# Autodesk Inventor assembly: Rear Crossbrace
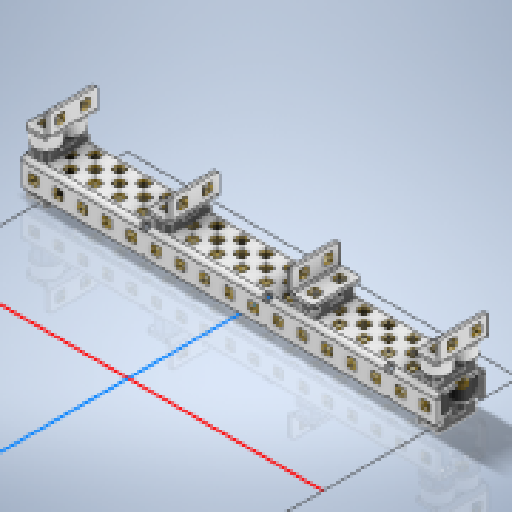
[picture p0: Inventor's stored thumbnail of the model, 512x512]
Saved by Autodesk Inventor 2026 (Build 300175000, 175)
## iProperties
Created: 2025-04-02
Part Number: Rear Crossbrace
Document SubType Name: Assembly
Designer: avere
Author: avere
## Documents named in this file (10)
- C:\Users\avere\OneDrive\Documents\VEX-CAD\V5-CAD\drivetrain\Braces\Rear Crossbrace.iam
- C:\Users\avere\OneDrive\Documents\VEX-CAD\VEX-CAD-Inventor\Structure\C Channel\Aluminum 1x2x1\Alu C 1x2x1x17.ipt
- C:\Users\avere\OneDrive\Documents\VEX-CAD\VEX-CAD-Inventor\Structure\Angle\Aluminum 1x1\Alu Angle 1x1x2.ipt
- C:\Users\avere\OneDrive\Documents\VEX-CAD\VEX-CAD-Inventor\Motion\Shaft LS\Bearing Flat - Cut.ipt
- C:\Users\avere\OneDrive\Documents\VEX-CAD\VEX-CAD-Inventor\Motion\Spacers\Spacer Nylon .375 OD\NSpacer .375 OD x .375.ipt
- C:\Users\avere\OneDrive\Documents\VEX-CAD\VEX-CAD-Inventor\Motion\Spacers\Spacer Nylon .375 OD.ipt
- C:\Users\avere\OneDrive\Documents\VEX-CAD\VEX-CAD-Inventor\Motion\Spacers\Washer Steel\SWasher .375 OD x .062500.ipt
- C:\Users\avere\OneDrive\Documents\VEX-CAD\VEX-CAD-Inventor\Motion\Spacers\Washer Steel.ipt
- C:\Users\avere\OneDrive\Documents\VEX-CAD\VEX-CAD-Inventor\Motion\Spacers\Spacer Nylon .500 OD\NSpacer White .500 OD x .250.ipt
- C:\Users\avere\OneDrive\Documents\VEX-CAD\VEX-CAD-Inventor\Motion\Spacers\Spacer Nylon .500 OD.ipt
## Components (23 placed, 6 different names)
1. Alu C 1x2x1x17:1 — Mate:1, Flush:1, Insert:1, Mate:4, Insert:12, Mate:7, Insert:22, Mate:10, Insert:30, Mate:16
2. Alu Angle 1x1x2:1 — Insert:2, Mate:3
3. Bearing Flat - Cut:1 — Insert:1, Insert:2, Mate:3, Mate:4
4. Alu Angle 1x1x2:2 — Mate:5, Insert:3, Mate:6
5. Bearing Flat - Cut:2 — Mate:5, Insert:3, Mate:6
6. Bearing Flat - Cut:3 — Insert:10, Insert:11
7. NSpacer .375 OD x .375:1 — Insert:8, Insert:10
8. SWasher .375 OD x .062500:1 — Insert:8, Insert:12
9. NSpacer .375 OD x .375:2 — Insert:9, Insert:11
10. SWasher .375 OD x .062500:2 — Insert:9, Mate:7
11. Bearing Flat - Cut:4 — Insert:13, Insert:14, Insert:17, Insert:18
12. NSpacer .375 OD x .375:3 — Insert:13, Insert:14, Insert:15, Insert:16
13. SWasher .375 OD x .062500:3 — Insert:15, Insert:16
14. NSpacer .375 OD x .375:4 — Insert:17, Insert:18, Insert:19, Insert:20
15. SWasher .375 OD x .062500:4 — Insert:19, Insert:20
16. Alu Angle 1x1x2:3 — Insert:31, Mate:17
17. Bearing Flat - Cut:5 — Insert:22, Mate:10, Insert:25, Insert:26
18. NSpacer White .500 OD x .250:1 — Insert:25, Mate:17
19. NSpacer White .500 OD x .250:2 — Insert:26, Insert:31
20. Alu Angle 1x1x2:5 — Insert:27, Mate:14, Mate:15
21. Bearing Flat - Cut:7 — Insert:27, Mate:14, Mate:15, Insert:28, Insert:29, Insert:30
22. NSpacer White .500 OD x .250:3 — Insert:28, Mate:16
23. NSpacer White .500 OD x .250:4 — Insert:29
## Relationships (41: Insert 28, Mate 12, Flush 1)
- Mate:1 (50.8 mm): Alu C 1x2x1x17:1
- Flush:1 (-107.95 mm): Alu C 1x2x1x17:1
- [Mate]: Alu Angle 1x1x2:1 ↔ Bearing Flat - Cut:1
- Insert:1: Alu C 1x2x1x17:1 ↔ Bearing Flat - Cut:1
- Insert:2: Alu Angle 1x1x2:1 ↔ Bearing Flat - Cut:1
- Mate:3: Alu Angle 1x1x2:1 ↔ Bearing Flat - Cut:1
- Mate:4: Alu C 1x2x1x17:1 ↔ Bearing Flat - Cut:1
- Mate:5: Alu Angle 1x1x2:2 ↔ Bearing Flat - Cut:2
- Insert:3: Alu Angle 1x1x2:2 ↔ Bearing Flat - Cut:2
- Mate:6: Alu Angle 1x1x2:2 ↔ Bearing Flat - Cut:2
- [Insert]: NSpacer .375 OD x .375:1 ↔ SWasher .375 OD x .062500:1
- [Insert]: Bearing Flat - Cut:3 ↔ NSpacer .375 OD x .375:1
- [Insert]: NSpacer .375 OD x .375:2 ↔ SWasher .375 OD x .062500:2
- [Insert]: Bearing Flat - Cut:3 ↔ NSpacer .375 OD x .375:2
- Insert:8: NSpacer .375 OD x .375:1 ↔ SWasher .375 OD x .062500:1
- Insert:9: NSpacer .375 OD x .375:2 ↔ SWasher .375 OD x .062500:2
- Insert:10: Bearing Flat - Cut:3 ↔ NSpacer .375 OD x .375:1
- Insert:11: Bearing Flat - Cut:3 ↔ NSpacer .375 OD x .375:2
- Insert:12: Alu C 1x2x1x17:1 ↔ SWasher .375 OD x .062500:1
- Mate:7: Alu C 1x2x1x17:1 ↔ SWasher .375 OD x .062500:2
- Insert:13: Bearing Flat - Cut:4 ↔ NSpacer .375 OD x .375:3
- Insert:14: Bearing Flat - Cut:4 ↔ NSpacer .375 OD x .375:3
- Insert:15: NSpacer .375 OD x .375:3 ↔ SWasher .375 OD x .062500:3
- Insert:16: NSpacer .375 OD x .375:3 ↔ SWasher .375 OD x .062500:3
- Insert:17: Bearing Flat - Cut:4 ↔ NSpacer .375 OD x .375:4
- Insert:18: Bearing Flat - Cut:4 ↔ NSpacer .375 OD x .375:4
- Insert:19: NSpacer .375 OD x .375:4 ↔ SWasher .375 OD x .062500:4
- Insert:20: NSpacer .375 OD x .375:4 ↔ SWasher .375 OD x .062500:4
- Insert:22: Alu C 1x2x1x17:1 ↔ Bearing Flat - Cut:5
- Mate:10: Alu C 1x2x1x17:1 ↔ Bearing Flat - Cut:5
- Insert:25: Bearing Flat - Cut:5 ↔ NSpacer White .500 OD x .250:1
- Insert:26: Bearing Flat - Cut:5 ↔ NSpacer White .500 OD x .250:2
- Insert:27 (6.35 mm): Alu Angle 1x1x2:5 ↔ Bearing Flat - Cut:7
- Mate:14: Alu Angle 1x1x2:5 ↔ Bearing Flat - Cut:7
- Mate:15: Alu Angle 1x1x2:5 ↔ Bearing Flat - Cut:7
- Insert:28: Bearing Flat - Cut:7 ↔ NSpacer White .500 OD x .250:3
- Insert:29: Bearing Flat - Cut:7 ↔ NSpacer White .500 OD x .250:4
- Insert:30: Alu C 1x2x1x17:1 ↔ Bearing Flat - Cut:7
- Mate:16: Alu C 1x2x1x17:1 ↔ NSpacer White .500 OD x .250:3
- Insert:31: Alu Angle 1x1x2:3 ↔ NSpacer White .500 OD x .250:2
- Mate:17: Alu Angle 1x1x2:3 ↔ NSpacer White .500 OD x .250:1
## Named parameters: d12_d11 = 0 mm, d13_d11 = 0 mm
